# Autodesk Inventor assembly: A2017_T4_13
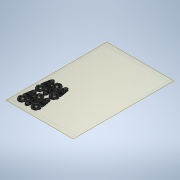
[picture p0: Inventor's stored thumbnail of the model, 180x180]
Saved by Autodesk Inventor 2020 (Build 240168000, 168)
## iProperties
Created: 2021-08-27
Part Number: A2017_T4_13
Document SubType Name: Assembly
Designer: Masato
Author: Masato
## Documents named in this file (3)
- C:\Users\naoki\Documents\Inventor\CitBrains\git_clone\SUSTAINA_ver1_0\220624_T4_13\SUSTAINA-OP\Cam\A2017_T4_13.iam
- C:\Users\naoki\Documents\Inventor\CitBrains\git_clone\SUSTAINA_ver1_0\220624_T4_13\SUSTAINA-OP\Cam\DisposableBoard.ipt
- C:\Users\naoki\Documents\Inventor\CitBrains\git_clone\SUSTAINA_ver1_0\220624_T4_13\SUSTAINA-OP\LowerBody\Ankle\Ankle_side_pitch_frame.ipt
## Components (7 placed, 2 different names)
1. DisposableBoard:1 — メイト:2, メイト:1, フラッシュ:1, フラッシュ:2, メイト:12, メイト:13, メイト:14, 正接:1, 正接:2, 正接:3, 正接:4
2. Ankle_side_pitch_frame:1 — メイト:12, 角度:1, メイト:15, 正接:1, 正接:4
3. Ankle_side_pitch_frame:2 — メイト:13, メイト:15, メイト:16, 正接:2
4. Ankle_side_pitch_frame:3 — メイト:14, メイト:16, 正接:3
5. Ankle_side_pitch_frame:4
6. Ankle_side_pitch_frame:5
7. Ankle_side_pitch_frame:6
## Component patterns: (2 elements, first: Ankle_side_pitch_frame:1 + Ankle_side_pitch_frame:2 + Ankle_side_pitch_frame:3)
## Relationships (14: Mate 7, Tangent 4, Flush 2, Angle 1)
- メイト:2 [Mate]: DisposableBoard:1
- メイト:1 [Mate]: DisposableBoard:1
- フラッシュ:1 [Flush]: DisposableBoard:1
- フラッシュ:2 [Flush]: DisposableBoard:1
- メイト:12 [Mate]: DisposableBoard:1 ↔ Ankle_side_pitch_frame:1
- メイト:13 [Mate]: DisposableBoard:1 ↔ Ankle_side_pitch_frame:2
- メイト:14 [Mate]: DisposableBoard:1 ↔ Ankle_side_pitch_frame:3
- 角度:1 [Angle] (90 deg): Ankle_side_pitch_frame:1
- メイト:15 [Mate] (2.5 mm): Ankle_side_pitch_frame:1 ↔ Ankle_side_pitch_frame:2
- メイト:16 [Mate] (2.5 mm): Ankle_side_pitch_frame:2 ↔ Ankle_side_pitch_frame:3
- 正接:1 [Tangent] (2 mm): DisposableBoard:1 ↔ Ankle_side_pitch_frame:1
- 正接:2 [Tangent] (2 mm): DisposableBoard:1 ↔ Ankle_side_pitch_frame:2
- 正接:3 [Tangent] (2 mm): DisposableBoard:1 ↔ Ankle_side_pitch_frame:3
- 正接:4 [Tangent] (2 mm): DisposableBoard:1 ↔ Ankle_side_pitch_frame:1
